# Autodesk Inventor assembly: tester
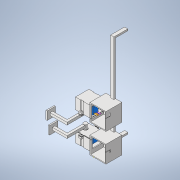
[picture p0: Inventor's stored thumbnail of the model, 180x180]
Saved by Autodesk Inventor 2020.2 (Build 242310000, 310)
## iProperties
Created: 2020-02-05
Part Number: tester
Document SubType Name: Assembly
Designer: ColinP
Author: ColinP
## Documents named in this file (6)
- C:\Users\ColinP\Documents\Inventor\steppermotoriqc\SteppermotorLaser\tester.iam
- C:\Users\ColinP\Documents\Inventor\steppermotoriqc\28BYJ-48 – 5V Stepper Motor\28BYJ-48 – 5V Stepper Motor.ipt
- C:\Users\ColinP\Documents\Inventor\steppermotoriqc\SteppermotorLaser\lid 4.0.ipt
- C:\Users\ColinP\Documents\Inventor\steppermotoriqc\SteppermotorLaser\shell 6.0.ipt
- C:\Users\ColinP\Documents\Inventor\steppermotoriqc\SteppermotorLaser\socket.ipt
- C:\Users\ColinP\Documents\Inventor\steppermotoriqc\SteppermotorLaser\socket2.ipt
## Components (7 placed, 5 different names)
1. 28BYJ-48 – 5V Stepper Motor:1 — Mate:1, Mate:2, Mate:3, Mate:4, Mate:5, Mate:17, Mate:18
2. lid 4.0:1 — Mate:4, Mate:5, Mate:6
3. 28BYJ-48 – 5V Stepper Motor:2 — Mate:9, Mate:10, Mate:11, Mate:15, Mate:16
4. lid 4.0:2 — Mate:12, Mate:13, Mate:14
5. socket:1 — Mate:15, Mate:16
6. socket2:1 — Mate:17, Mate:18
7. shell 6.0:1 — Mate:1, Mate:2, Mate:3, Mate:6, Mate:9, Mate:10, Mate:11, Mate:12, Mate:13, Mate:14
## Relationships (16: Mate 16)
- Mate:1: 28BYJ-48 – 5V Stepper Motor:1 ↔ shell 6.0:1
- Mate:2: 28BYJ-48 – 5V Stepper Motor:1 ↔ shell 6.0:1
- Mate:3: 28BYJ-48 – 5V Stepper Motor:1 ↔ shell 6.0:1
- Mate:4: 28BYJ-48 – 5V Stepper Motor:1 ↔ lid 4.0:1
- Mate:5: 28BYJ-48 – 5V Stepper Motor:1 ↔ lid 4.0:1
- Mate:6: lid 4.0:1 ↔ shell 6.0:1
- Mate:9: 28BYJ-48 – 5V Stepper Motor:2 ↔ shell 6.0:1
- Mate:10: 28BYJ-48 – 5V Stepper Motor:2 ↔ shell 6.0:1
- Mate:11: 28BYJ-48 – 5V Stepper Motor:2 ↔ shell 6.0:1
- Mate:12: lid 4.0:2 ↔ shell 6.0:1
- Mate:13: lid 4.0:2 ↔ shell 6.0:1
- Mate:14: lid 4.0:2 ↔ shell 6.0:1
- Mate:15: 28BYJ-48 – 5V Stepper Motor:2 ↔ socket:1
- Mate:16: 28BYJ-48 – 5V Stepper Motor:2 ↔ socket:1
- Mate:17: 28BYJ-48 – 5V Stepper Motor:1 ↔ socket2:1
- Mate:18: 28BYJ-48 – 5V Stepper Motor:1 ↔ socket2:1
